# Autodesk Inventor assembly: robotnoturret
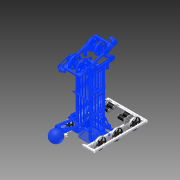
[picture p0: Inventor's stored thumbnail of the model, 180x180]
Saved by Autodesk Inventor 2011 SP1 (Build 150282100, 282)
## iProperties
Created: 2012-01-20
Part Number: robotnoturret
Document SubType Name: Assembly
Designer: Christopher
Author: Christopher
## Documents named in this file (3)
- C:\Users\Christopher\Documents\Christopher\FIRST\Inventor files\2012\non-pivot shooter\robotnoturret.iam
- C:\Users\Christopher\Documents\Christopher\FIRST\Inventor files\2012\non-pivot shooter\towerbottomnorotate2.5.iam
- C:\Users\Christopher\Documents\Christopher\FIRST\Inventor files\2012\robot base.iam
## Components (2 placed, 2 different names)
1. towerbottomnorotate2.5:1 [sub-assembly] — Mate:1, Mate:2, Mate:3
2. robot base:1 [sub-assembly] — Mate:1, Mate:2, Mate:3
## Relationships (3: Mate 3)
- Mate:1: towerbottomnorotate2.5:1 ↔ robot base:1
- Mate:2: towerbottomnorotate2.5:1 ↔ robot base:1
- Mate:3 (127 mm): towerbottomnorotate2.5:1 ↔ robot base:1
